# Autodesk Inventor assembly: motorbrace
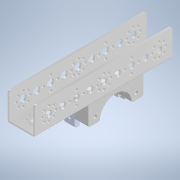
[picture p0: Inventor's stored thumbnail of the model, 180x180]
Saved by Autodesk Inventor 2020.1 (Build 241239000, 239)
## iProperties
Created: 2019-12-07
Part Number: motorbrace
Document SubType Name: Assembly
Designer: alpha
Author: alpha
## Documents named in this file (4)
- B:\Documents\GitHub\AO_Robotics\CAD\Projects\Joshua Schmidt\motorbrace.iam
- B:\Documents\GitHub\AO_Robotics\CAD\Parts Kits\FTC Tetrix KOP Organized (7-24-19)\Frame Hardware\Tetrix_39067.ipt
- B:\Documents\GitHub\AO_Robotics\CAD\Parts Kits\FTC Tetrix KOP Organized (7-24-19)\Motor\739376\Tetrix_739376_Base.ipt
- B:\Documents\AO print stuff\motorsupport.ipt
## Components (3 placed, 3 different names)
1. Tetrix_39067:1 — Rigid:1
2. Tetrix_739376_Base:1 — Rigid:1, Flush:1
3. motorsupport:1 — Flush:1
## Relationships (2: WeldJoint 1, Flush 1)
- Rigid:1 [WeldJoint]: Tetrix_39067:1 ↔ Tetrix_739376_Base:1
- Flush:1: Tetrix_739376_Base:1 ↔ motorsupport:1
